# Autodesk Inventor assembly: plolu z obudowa
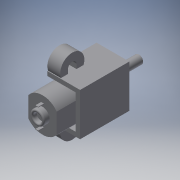
[picture p0: Inventor's stored thumbnail of the model, 180x180]
Saved by Autodesk Inventor 2016 (Build 200138000, 138)
## iProperties
Created: 2015-11-09
Part Number: plolu z obudowa
Material: Ogólny
Document SubType Name: Assembly
Designer: Mrianura
Author: Mrianura
## Documents named in this file (3)
- C:\Users\Mrianura\Documents\Inventor\katorga\plolu z obudowa.iam
- C:\Users\Mrianura\Desktop\Inventor - paczka czesci by Michal Burdka\pololu_of.ipt
- C:\Users\Mrianura\Documents\Inventor\katorga\przedluzone_mocowanie.ipt
## Components (2 placed, 2 different names)
1. pololu_of:1 — Sztywne:1
2. przedluzone_mocowanie:1 — Sztywne:1
## Relationships (1: WeldJoint 1)
- Sztywne:1 [WeldJoint]: pololu_of:1 ↔ przedluzone_mocowanie:1
